# Autodesk Inventor assembly: Tape Measure
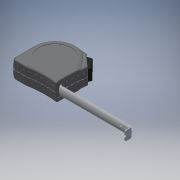
[picture p0: Inventor's stored thumbnail of the model, 180x180]
Saved by Autodesk Inventor 2019 (Build 230136000, 136)
## iProperties
Created: 2015-04-11
Part Number: Tape Measure
Description: STEP AP214
Document SubType Name: Assembly
Designer: Ashley
Sending System: SolidWorks 2015
Preprocessor: SwSTEP 2.0
Title: Tape Measure.STEP
Author: Hyper
Revision Number: HERHANGÝ
## Documents named in this file (12)
- C:\Users\Ashley\Desktop\repositories\design\inventor\2018-2019\Tape Measure.iam
- C:\Users\Ashley\Downloads\tape-measure-3.snapshot.9\Plastik Ürün 1.ipt
- C:\Users\Ashley\Downloads\tape-measure-3.snapshot.9\Makara.ipt
- C:\Users\Ashley\Downloads\tape-measure-3.snapshot.9\Plastik Ürün 2.ipt
- C:\Users\Ashley\Downloads\tape-measure-3.snapshot.9\Yaylý Plaka.ipt
- C:\Users\Ashley\Downloads\tape-measure-3.snapshot.9\Kitleme Tuþu.ipt
- C:\Users\Ashley\Downloads\tape-measure-3.snapshot.9\Þerit Cetvel.ipt
- C:\Users\Ashley\Downloads\tape-measure-3.snapshot.9\Kanca.ipt
- C:\Users\Ashley\Downloads\tape-measure-3.snapshot.9\Kanca Pimi.ipt
- C:\Users\Ashley\Downloads\tape-measure-3.snapshot.9\metre kanca.ipt
- C:\Users\Ashley\Downloads\tape-measure-3.snapshot.9\oval head_am_B18.6.7M - M2.5 x 0.45 x 20 Type I Cross Recessed OHMS --20C.ipt
- C:\Users\Ashley\Downloads\tape-measure-3.snapshot.9\oval head_am_B18.6.7M - M2.5 x 0.45 x 13 Type I Cross Recessed OHMS --13C.ipt
## Components (13 placed, 13 different names)
1. Plastik Ürün 1_1
2. Makara_2
3. Plastik Ürün 2_3
4. Yaylý Plaka_4
5. Kitleme Tuþu_5
6. Þerit Cetvel_6 — Mate:1
7. Kanca_7 — Mate:1
8. Kanca Pimi_8
9. Kanca Pimi_9
10. metre kanca_10
11. oval head_am_B18.6.7M - M2.5 x 0.45 x 20 Type I Cross Recessed OHMS --20C_11
12. oval head_am_B18.6.7M - M2.5 x 0.45 x 20 Type I Cross Recessed OHMS --20C_12
13. oval head_am_B18.6.7M - M2.5 x 0.45 x 13 Type I Cross Recessed OHMS --13C_13
## Relationships (1: Mate 1)
- Mate:1: Þerit Cetvel_6 ↔ Kanca_7
